# Autodesk Inventor assembly: mezzanineBoard
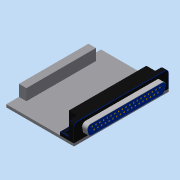
[picture p0: Inventor's stored thumbnail of the model, 180x180]
Saved by Autodesk Inventor 2016 (Build 200138000, 138)
## iProperties
Created: 2016-08-31
Part Number: mezzanineBoard
Document SubType Name: Assembly
Designer: Zara
Author: Zara
## Documents named in this file (4)
- C:\Users\Zara\Documents\hera-cad\Node\mezzanineBoard.iam
- C:\Users\Zara\Documents\hera-cad\Node\mezzaninePCB.ipt
- C:\Users\Zara\Downloads\db9-db15-db25-db37-connector (1)\DB37RA_Fz.ipt
- C:\Users\Zara\Documents\hera-cad\Node\snapPinout.ipt
## Components (3 placed, 3 different names)
1. mezzaninePCB:1 — Flush:1, Mate:1, Flush:2, Mate:2, Flush:3, Flush:4
2. DB37RA_Fz:1 — Flush:1, Mate:1, Flush:2
3. snapPinout:1 — Mate:2, Flush:3, Flush:4
## Relationships (6: Flush 4, Mate 2)
- Flush:1: mezzaninePCB:1 ↔ DB37RA_Fz:1
- Mate:1: mezzaninePCB:1 ↔ DB37RA_Fz:1
- Flush:2: mezzaninePCB:1 ↔ DB37RA_Fz:1
- Mate:2: mezzaninePCB:1 ↔ snapPinout:1
- Flush:3: mezzaninePCB:1 ↔ snapPinout:1
- Flush:4 (9.3 mm): mezzaninePCB:1 ↔ snapPinout:1
